# Autodesk Inventor assembly: Zespol1
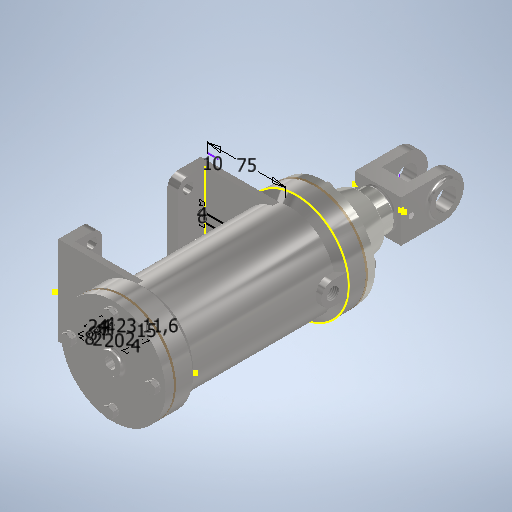
[picture p0: Inventor's stored thumbnail of the model, 512x512]
Saved by Autodesk Inventor 2025 (Build 290162000, 162)
## iProperties
Created: 2025-03-23
Part Number: Zespol1
Document SubType Name: Assembly
Designer: marci
Author: marci
## Documents named in this file (15)
- C:\Users\barte\Downloads\Zespol1 (1).iam
- C:\Users\barte\Downloads\01cylinder (2).ipt
- C:\Users\barte\OneDrive - Akademia Górniczo-Hutnicza im. Stanisława Staszica w Krakowie\Pulpit\proj1\02pokrywa.ipt
- C:\Users\barte\OneDrive - Akademia Górniczo-Hutnicza im. Stanisława Staszica w Krakowie\Pulpit\proj1\04tloczysko.ipt
- C:\Users\barte\OneDrive - Akademia Górniczo-Hutnicza im. Stanisława Staszica w Krakowie\Pulpit\proj1\7Tłok.ipt
- C:\Users\barte\OneDrive - Akademia Górniczo-Hutnicza im. Stanisława Staszica w Krakowie\Pulpit\proj1\08pokrywa (2).ipt
- C:\Users\barte\OneDrive - Akademia Górniczo-Hutnicza im. Stanisława Staszica w Krakowie\Pulpit\proj1\06widelki.ipt
- C:\Users\barte\OneDrive - Akademia Górniczo-Hutnicza im. Stanisława Staszica w Krakowie\Pulpit\proj1\Sprężyna naciskowa11.ipt
- C:\Users\barte\OneDrive - Akademia Górniczo-Hutnicza im. Stanisława Staszica w Krakowie\Pulpit\proj1\uszczelka.ipt
- C:\Users\barte\OneDrive - Akademia Górniczo-Hutnicza im. Stanisława Staszica w Krakowie\Pulpit\proj1\pierśnień.ipt
- C:\Users\barte\Downloads\kołek.ipt
- C:\Users\barte\Documents\Inventor\Content Center Files\R2025\pl-PL\PN-85 M-82101 A\PN-85_M-82101 - M 6 x 25 - 1(1).ipt
- C:\Users\barte\Downloads\2pokrywa.ipt
- C:\Users\barte\Documents\Inventor\Content Center Files\R2025\pl-PL\PN-78 M-82007\PN-78_M-82007 - 6,4.ipt
- C:\Users\barte\Downloads\04tloczysko (1).ipt
## Components (30 placed, 14 different names)
1. 01cylinder (2):1 — Obrotowe:4, Obrotowe:5, Obrotowe:6, Obrotowe:7, Sztywne:2
2. 02pokrywa:1 — Obrotowe:8
3. 7Tłok:1 — Obrotowe:1, Równoległe:1, Obrotowe:2, Obrotowe:3, Obrotowe:4
4. 08pokrywa (2):1 — Obrotowe:7, Obrotowe:17, Obrotowe:29, Obrotowe:30, Obrotowe:31, Obrotowe:32
5. 06widelki:1 — Obrotowe:17, Obrotowe:18
6. 04tloczysko:1 — Obrotowe:1, Zestawiające:1
7. Sprężyna naciskowa1:2 — Zestawiające:1, Równoległe:1
8. uszczelka:1 — Obrotowe:6, Obrotowe:8, Obrotowe:19
9. uszczelka:2 — Obrotowe:5
10. pierśnień:1 — Obrotowe:2
11. pierśnień:2 — Obrotowe:3
12. kołek:1 — Obrotowe:18
13. PN-85/M-82101 Klasa A M 6 x 25:1 — Obrotowe:28
14. PN-85/M-82101 Klasa A M 6 x 25:2 — Obrotowe:25
15. PN-85/M-82101 Klasa A M 6 x 25:3 — Obrotowe:26
16. PN-85/M-82101 Klasa A M 6 x 25:4 — Obrotowe:27
17. PN-85/M-82101 Klasa A M 6 x 25:5 — Obrotowe:34
18. PN-85/M-82101 Klasa A M 6 x 25:6 — Obrotowe:35
19. PN-85/M-82101 Klasa A M 6 x 25:7 — Obrotowe:36
20. PN-85/M-82101 Klasa A M 6 x 25:8 — Obrotowe:33
21. 2pokrywa:1 — Obrotowe:19, Sztywne:1, Obrotowe:22, Obrotowe:23, Obrotowe:24
22. PN-78/M-82007 6,4:2 — Obrotowe:22, Obrotowe:26
23. PN-78/M-82007 6,4:3 — Sztywne:1, Obrotowe:25
24. PN-78/M-82007 6,4:4 — Obrotowe:23, Obrotowe:27
25. PN-78/M-82007 6,4:5 — Obrotowe:29, Obrotowe:33
26. PN-78/M-82007 6,4:6 — Obrotowe:24, Obrotowe:28
27. PN-78/M-82007 6,4:7 — Obrotowe:30, Obrotowe:34
28. PN-78/M-82007 6,4:8 — Obrotowe:31, Obrotowe:36
29. PN-78/M-82007 6,4:9 — Obrotowe:32, Obrotowe:35
30. 04tloczysko (1):2 — Sztywne:2
## Relationships (30: RevoluteJoint 26, WeldJoint 2, Mate 1, Flush 1)
- Obrotowe:1 [RevoluteJoint]: 7Tłok:1 ↔ 04tloczysko:1
- Zestawiające:1 [Mate]: 04tloczysko:1 ↔ Sprężyna naciskowa1:2
- Równoległe:1 [Flush]: 7Tłok:1 ↔ Sprężyna naciskowa1:2
- Obrotowe:2 [RevoluteJoint]: 7Tłok:1 ↔ pierśnień:1
- Obrotowe:3 [RevoluteJoint]: 7Tłok:1 ↔ pierśnień:2
- Obrotowe:4 [RevoluteJoint]: 01cylinder (2):1 ↔ 7Tłok:1
- Obrotowe:5 [RevoluteJoint]: 01cylinder (2):1 ↔ uszczelka:2
- Obrotowe:6 [RevoluteJoint]: 01cylinder (2):1 ↔ uszczelka:1
- Obrotowe:7 [RevoluteJoint]: 01cylinder (2):1 ↔ 08pokrywa (2):1
- Obrotowe:8 [RevoluteJoint]: 02pokrywa:1 ↔ uszczelka:1
- Obrotowe:17 [RevoluteJoint]: 08pokrywa (2):1 ↔ 06widelki:1
- Obrotowe:18 [RevoluteJoint]: 06widelki:1 ↔ kołek:1
- Obrotowe:19 [RevoluteJoint]: uszczelka:1 ↔ 2pokrywa:1
- Sztywne:1 [WeldJoint]: 2pokrywa:1 ↔ PN-78/M-82007 6,4:3
- Obrotowe:22 [RevoluteJoint]: 2pokrywa:1 ↔ PN-78/M-82007 6,4:2
- Obrotowe:23 [RevoluteJoint]: 2pokrywa:1 ↔ PN-78/M-82007 6,4:4
- Obrotowe:24 [RevoluteJoint]: 2pokrywa:1 ↔ PN-78/M-82007 6,4:6
- Obrotowe:25 [RevoluteJoint]: PN-85/M-82101 Klasa A M 6 x 25:2 ↔ PN-78/M-82007 6,4:3
- Obrotowe:26 [RevoluteJoint]: PN-85/M-82101 Klasa A M 6 x 25:3 ↔ PN-78/M-82007 6,4:2
- Obrotowe:27 [RevoluteJoint]: PN-85/M-82101 Klasa A M 6 x 25:4 ↔ PN-78/M-82007 6,4:4
- Obrotowe:28 [RevoluteJoint]: PN-85/M-82101 Klasa A M 6 x 25:1 ↔ PN-78/M-82007 6,4:6
- Obrotowe:29 [RevoluteJoint]: 08pokrywa (2):1 ↔ PN-78/M-82007 6,4:5
- Obrotowe:30 [RevoluteJoint]: 08pokrywa (2):1 ↔ PN-78/M-82007 6,4:7
- Obrotowe:31 [RevoluteJoint]: 08pokrywa (2):1 ↔ PN-78/M-82007 6,4:8
- Obrotowe:32 [RevoluteJoint]: 08pokrywa (2):1 ↔ PN-78/M-82007 6,4:9
- Obrotowe:33 [RevoluteJoint]: PN-85/M-82101 Klasa A M 6 x 25:8 ↔ PN-78/M-82007 6,4:5
- Obrotowe:34 [RevoluteJoint]: PN-85/M-82101 Klasa A M 6 x 25:5 ↔ PN-78/M-82007 6,4:7
- Obrotowe:35 [RevoluteJoint]: PN-85/M-82101 Klasa A M 6 x 25:6 ↔ PN-78/M-82007 6,4:9
- Obrotowe:36 [RevoluteJoint]: PN-85/M-82101 Klasa A M 6 x 25:7 ↔ PN-78/M-82007 6,4:8
- Sztywne:2 [WeldJoint]: 01cylinder (2):1 ↔ 04tloczysko (1):2
